# Autodesk Inventor assembly: nc_nhk7
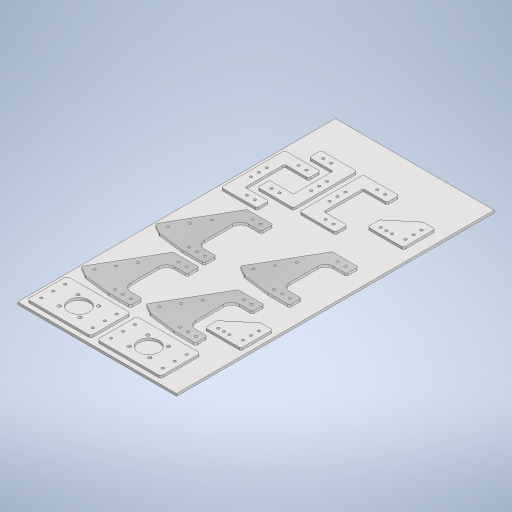
[picture p0: Inventor's stored thumbnail of the model, 512x512]
Saved by Autodesk Inventor 2023 (Build 270158000, 158)
## iProperties
Created: 2022-04-20
Part Number: nc_nhk7
Document SubType Name: Assembly
Designer: yuta
Author: yuta
## Documents named in this file (6)
- C:\Users\yuta\Documents\NHK\nc_nhk7.iam
- C:\Users\yuta\Documents\NHK\NC.port.ipt
- C:\Users\yuta\Documents\NHK\射出_モーター固定1.ipt
- C:\Users\yuta\Desktop\オムニホイール\ホイールユニット_側板1.ipt
- C:\Users\yuta\Documents\NHK\射出_固定3.ipt
- C:\Users\yuta\Documents\NHK\射出_固定1.ipt
## Components (12 placed, 5 different names)
1. NC.port:1 — メイト:1, フラッシュ:1, フラッシュ:2, メイト:2, フラッシュ:3, メイト:4, メイト:6, メイト:7, メイト:10, メイト:12, メイト:13, メイト:14, フラッシュ:4, メイト:19, フラッシュ:5, メイト:21, メイト:24, メイト:26
2. 射出_モーター固定1:1 — メイト:1, フラッシュ:1, フラッシュ:2, メイト:3, メイト:5
3. 射出_モーター固定1:2 — メイト:2, メイト:3, フラッシュ:3, メイト:8
4. ホイールユニット_側板1:1 — メイト:13
5. ホイールユニット_側板1:2 — メイト:4, メイト:5, メイト:6, メイト:9, メイト:11
6. ホイールユニット_側板1:3 — メイト:10, メイト:11, メイト:12, メイト:20
7. ホイールユニット_側板1:4 — メイト:7, メイト:8, メイト:9, メイト:15
8. 射出_固定3:1 — メイト:14, フラッシュ:4, メイト:15
9. 射出_固定1:1 — メイト:19, フラッシュ:5, メイト:20, メイト:22, メイト:23
10. 射出_固定1:2 — メイト:21, メイト:22, メイト:23, メイト:25, フラッシュ:6
11. 射出_固定1:4 — メイト:24, メイト:25, フラッシュ:6
12. 射出_固定3:2 — メイト:26
## Relationships (29: Mate 23, Flush 6)
- メイト:1 [Mate]: NC.port:1 ↔ 射出_モーター固定1:1
- フラッシュ:1 [Flush] (6 mm): NC.port:1 ↔ 射出_モーター固定1:1
- フラッシュ:2 [Flush] (6 mm): NC.port:1 ↔ 射出_モーター固定1:1
- メイト:2 [Mate]: NC.port:1 ↔ 射出_モーター固定1:2
- メイト:3 [Mate] (8 mm): 射出_モーター固定1:1 ↔ 射出_モーター固定1:2
- フラッシュ:3 [Flush] (6 mm): NC.port:1 ↔ 射出_モーター固定1:2
- メイト:4 [Mate]: NC.port:1 ↔ ホイールユニット_側板1:2
- メイト:5 [Mate] (8 mm): 射出_モーター固定1:1 ↔ ホイールユニット_側板1:2
- メイト:6 [Mate] (-7 mm): NC.port:1 ↔ ホイールユニット_側板1:2
- メイト:7 [Mate]: NC.port:1 ↔ ホイールユニット_側板1:4
- メイト:8 [Mate] (8 mm): 射出_モーター固定1:2 ↔ ホイールユニット_側板1:4
- メイト:9 [Mate] (11 mm): ホイールユニット_側板1:2 ↔ ホイールユニット_側板1:4
- メイト:10 [Mate]: NC.port:1 ↔ ホイールユニット_側板1:3
- メイト:11 [Mate] (8 mm): ホイールユニット_側板1:2 ↔ ホイールユニット_側板1:3
- メイト:12 [Mate] (-7 mm): NC.port:1 ↔ ホイールユニット_側板1:3
- メイト:13 [Mate]: NC.port:1 ↔ ホイールユニット_側板1:1
- メイト:14 [Mate]: NC.port:1 ↔ 射出_固定3:1
- フラッシュ:4 [Flush] (6 mm): NC.port:1 ↔ 射出_固定3:1
- メイト:15 [Mate] (8 mm): ホイールユニット_側板1:4 ↔ 射出_固定3:1
- メイト:19 [Mate]: NC.port:1 ↔ 射出_固定1:1
- フラッシュ:5 [Flush] (6 mm): NC.port:1 ↔ 射出_固定1:1
- メイト:20 [Mate] (8 mm): ホイールユニット_側板1:3 ↔ 射出_固定1:1
- メイト:21 [Mate]: NC.port:1 ↔ 射出_固定1:2
- メイト:22 [Mate] (8 mm): 射出_固定1:1 ↔ 射出_固定1:2
- メイト:23 [Mate] (8 mm): 射出_固定1:1 ↔ 射出_固定1:2
- メイト:24 [Mate]: NC.port:1 ↔ 射出_固定1:4
- メイト:25 [Mate] (8 mm): 射出_固定1:2 ↔ 射出_固定1:4
- フラッシュ:6 [Flush]: 射出_固定1:2 ↔ 射出_固定1:4
- メイト:26 [Mate]: NC.port:1 ↔ 射出_固定3:2
